# Autodesk Inventor assembly: Assembly1
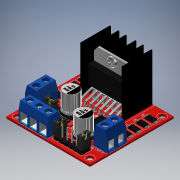
[picture p0: Inventor's stored thumbnail of the model, 180x180]
Saved by Autodesk Inventor 2019 (Build 230136000, 136)
## iProperties
Created: 2022-10-14
Part Number: Assembly1
Document SubType Name: Assembly
Designer: Tecneu
Author: Tecneu
## Documents named in this file (3)
- C:\Users\Tecneu\Documents\ZD\Modelos 3D\Puente H L298\Assembly1.iam
- C:\Users\Tecneu\Documents\ZD\Modelos 3D\Puente H L298\Part1_l298.ipt
- C:\Users\Tecneu\Documents\ZD\Modelos 3D\Puente H L298\Jumper.ipt
## Components (4 placed, 2 different names)
1. Part1_l298:1 — Flush:1, Flush:2, Flush:3, Mate:1, Mate:2, Mate:3, Mate:4, Mate:5, Mate:6, Mate:7, Mate:8, Mate:9
2. Jumper:2 — Mate:4, Mate:5, Mate:6
3. Jumper:3 — Mate:1, Mate:2, Mate:3
4. Jumper:4 — Mate:7, Mate:8, Mate:9
## Relationships (12: Mate 9, Flush 3)
- Flush:1: Part1_l298:1
- Flush:2: Part1_l298:1
- Flush:3: Part1_l298:1
- Mate:1: Part1_l298:1 ↔ Jumper:3
- Mate:2 (0.3 mm): Part1_l298:1 ↔ Jumper:3
- Mate:3 (0.02 mm): Part1_l298:1 ↔ Jumper:3
- Mate:4: Part1_l298:1 ↔ Jumper:2
- Mate:5 (0.5 mm): Part1_l298:1 ↔ Jumper:2
- Mate:6 (0.03 mm): Part1_l298:1 ↔ Jumper:2
- Mate:7: Part1_l298:1 ↔ Jumper:4
- Mate:8 (0.03 mm): Part1_l298:1 ↔ Jumper:4
- Mate:9 (0.3 mm): Part1_l298:1 ↔ Jumper:4
